# Autodesk Inventor assembly: MotorMount_Main
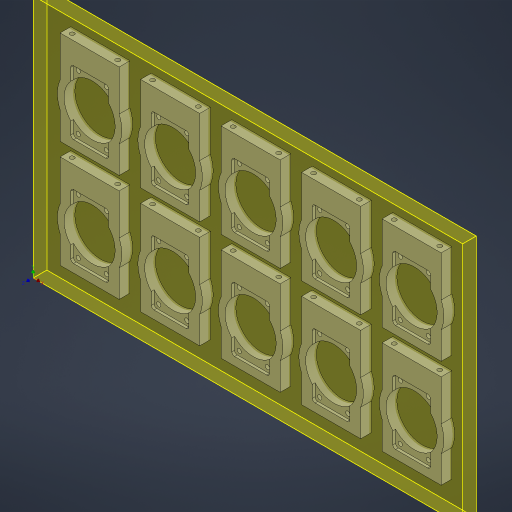
[picture p0: Inventor's stored thumbnail of the model, 512x512]
Saved by Autodesk Inventor 2024.2 (Build 282272000, 272)
## iProperties
Created: 2023-12-28
Part Number: MotorMount_Main
Document SubType Name: Assembly
Designer: Hanaoka
Author: Hanaoka
## Documents named in this file (2)
- G:\共有ドライブ\reRo\05_個人\hanaoka\inventor\CAMpath\MotorMount_Main.iam
- G:\共有ドライブ\reRo\05_個人\hanaoka\inventor\DriveUnit\MotorMount_main.ipt
## Components (10 placed, 1 different names)
1. MotorMount_main:1 — メイト:1, メイト:2, メイト:3
2. MotorMount_main:2
3. MotorMount_main:3
4. MotorMount_main:4
5. MotorMount_main:5
6. MotorMount_main:6
7. MotorMount_main:7
8. MotorMount_main:8
9. MotorMount_main:9
10. MotorMount_main:10
## Component patterns: (10 elements, first: MotorMount_main:1)
## Relationships (3: Mate 3)
- メイト:1 [Mate]: MotorMount_main:1
- メイト:2 [Mate]: MotorMount_main:1
- メイト:3 [Mate]: MotorMount_main:1
